# Autodesk Inventor assembly: Assembly1
(part 2 of 3)
- Mate:224: Plattform-Oberteil:1 ↔ DIN 125-1 B B 6,4:8
- Mate:225: Plattform-Oberteil:1 ↔ DIN 931-1 - replaced by DIN EN 24014 M6 x 30:4
- Mate:226: Plattform-Oberteil:1 ↔ DIN 931-1 - replaced by DIN EN 24014 M6 x 30:14
- Mate:227: Plattform-Oberteil:1 ↔ DIN 931-1 - replaced by DIN EN 24014 M6 x 30:5
- Mate:228: DIN 931-1 - replaced by DIN EN 24014 M8 x 45:1 ↔ DIN 125-1 B B 8,4:1
- Mate:229: DIN 931-1 - replaced by DIN EN 24014 M8 x 45:1 ↔ DIN 125-1 B B 8,4:1
- [Mate]: DIN 931-1 - replaced by DIN EN 24014 M8 x 45:2 ↔ DIN 125-1 B B 8,4:2
- [Mate]: DIN 931-1 - replaced by DIN EN 24014 M8 x 45:2 ↔ DIN 125-1 B B 8,4:2
- [Mate]: DIN 931-1 - replaced by DIN EN 24014 M8 x 45:3 ↔ DIN 125-1 B B 8,4:3
- [Mate]: DIN 931-1 - replaced by DIN EN 24014 M8 x 45:3 ↔ DIN 125-1 B B 8,4:3
- [Mate]: DIN 931-1 - replaced by DIN EN 24014 M8 x 45:4 ↔ DIN 125-1 B B 8,4:4
- [Mate]: DIN 931-1 - replaced by DIN EN 24014 M8 x 45:4 ↔ DIN 125-1 B B 8,4:4
- Mate:236: Plattform-Unterteil:1 ↔ DIN 125-1 B B 8,4:1
- Mate:237: Plattform-Unterteil:1 ↔ DIN 125-1 B B 8,4:4
- Mate:238: Plattform-Unterteil:1 ↔ DIN 125-1 B B 8,4:2
- Mate:239: Plattform-Unterteil:1 ↔ DIN 125-1 B B 8,4:3
- Mate:240: Verbindungsplatte:1 ↔ DIN 931-1 - replaced by DIN EN 24014 M8 x 45:3
- Mate:241: Verbindungsplatte:1 ↔ DIN 931-1 - replaced by DIN EN 24014 M8 x 45:4
- Mate:242: Plattform-Unterteil:1 ↔ DIN 931-1 - replaced by DIN EN 24014 M8 x 45:2
- Mate:243: Plattform-Unterteil:1 ↔ DIN 931-1 - replaced by DIN EN 24014 M8 x 45:1
- [Mate]: DIN 931-1 - replaced by DIN EN 24014 M8 x 50:5 ↔ DIN 125-1 B B 8,4:5
- [Mate]: DIN 931-1 - replaced by DIN EN 24014 M8 x 50:5 ↔ DIN 125-1 B B 8,4:5
- [Mate]: DIN 931-1 - replaced by DIN EN 24014 M8 x 50:6 ↔ DIN 125-1 B B 8,4:6
- [Mate]: DIN 931-1 - replaced by DIN EN 24014 M8 x 50:6 ↔ DIN 125-1 B B 8,4:6
- [Mate]: DIN 931-1 - replaced by DIN EN 24014 M8 x 50:7 ↔ DIN 125-1 B B 8,4:7
- [Mate]: DIN 931-1 - replaced by DIN EN 24014 M8 x 50:7 ↔ DIN 125-1 B B 8,4:7
- [Mate]: DIN 931-1 - replaced by DIN EN 24014 M8 x 50:8 ↔ DIN 125-1 B B 8,4:8
- [Mate]: DIN 931-1 - replaced by DIN EN 24014 M8 x 50:8 ↔ DIN 125-1 B B 8,4:8
- Mate:252: Verbindungsplatte:1 ↔ DIN 125-1 B B 8,4:8
- Mate:253: Verbindungsplatte:1 ↔ DIN 125-1 B B 8,4:7
- Mate:254: Verbindungsplatte:1 ↔ DIN 125-1 B B 8,4:6
- Mate:255: Verbindungsplatte:1 ↔ DIN 125-1 B B 8,4:5
- Mate:256: Verbindungsplatte:1 ↔ DIN 931-1 - replaced by DIN EN 24014 M8 x 50:8
- Mate:257: Verbindungsplatte:1 ↔ DIN 931-1 - replaced by DIN EN 24014 M8 x 50:7
- Mate:258: Verbindungsplatte:1 ↔ DIN 931-1 - replaced by DIN EN 24014 M8 x 50:6
- Mate:259: Verbindungsplatte:1 ↔ DIN 931-1 - replaced by DIN EN 24014 M8 x 50:5
- [Mate]: DIN 931-1 - replaced by DIN EN 24014 M6 x 50:3 ↔ DIN 125-1 B B 6,4:23
- [Mate]: DIN 931-1 - replaced by DIN EN 24014 M6 x 50:3 ↔ DIN 125-1 B B 6,4:23
- [Mate]: DIN 931-1 - replaced by DIN EN 24014 M6 x 50:2 ↔ DIN 125-1 B B 6,4:21
- [Mate]: DIN 931-1 - replaced by DIN EN 24014 M6 x 50:2 ↔ DIN 125-1 B B 6,4:21
- [Mate]: DIN 931-1 - replaced by DIN EN 24014 M6 x 50:1 ↔ DIN 125-1 B B 6,4:22
- [Mate]: DIN 931-1 - replaced by DIN EN 24014 M6 x 50:1 ↔ DIN 125-1 B B 6,4:22
- Mate:266: Deckel:1 ↔ DIN 125-1 B B 6,4:21
- Mate:267: Deckel:1 ↔ DIN 125-1 B B 6,4:22
- Mate:268: Deckel:1 ↔ DIN 125-1 B B 6,4:23
- Mate:269: Deckel:1 ↔ DIN 931-1 - replaced by DIN EN 24014 M6 x 50:2
- Mate:270: Deckel:1 ↔ DIN 931-1 - replaced by DIN EN 24014 M6 x 50:3
- Mate:271: Deckel:1 ↔ DIN 931-1 - replaced by DIN EN 24014 M6 x 50:1
- Mate:272: Festlagertopf:1 ↔ DIN 931-1 - replaced by DIN EN 24014 M6 x 50:2
- [Mate]: DIN 931-1 - replaced by DIN EN 24014 M5 x 25:1 ↔ DIN 125-1 B B 5,3:2
- [Mate]: DIN 931-1 - replaced by DIN EN 24014 M5 x 25:1 ↔ DIN 125-1 B B 5,3:2
- Mate:275: Verfahrschlitten:1 ↔ Gewindemutter:1
- Mate:276: Verfahrschlitten:1 ↔ Gewindemutter:1
- Mate:277: Verfahrschlitten:1 ↔ Gewindemutter:2
- Mate:278: Verfahrschlitten:1 ↔ Gewindemutter:2
- Mate:279: Verfahrschlitten:1 ↔ DIN 931-1 - replaced by DIN EN 24014 M5 x 25:1
- Mate:280: DIN 125-1 B B 5,3:2 ↔ Gewindemutter:1
- [Mate]: DIN 931-1 - replaced by DIN EN 24014 M5 x 25:2 ↔ DIN 125-1 B B 5,3:3
- [Mate]: DIN 931-1 - replaced by DIN EN 24014 M5 x 25:2 ↔ DIN 125-1 B B 5,3:3
- [Mate]: DIN 931-1 - replaced by DIN EN 24014 M5 x 25:3 ↔ DIN 125-1 B B 5,3:4
- [Mate]: DIN 931-1 - replaced by DIN EN 24014 M5 x 25:3 ↔ DIN 125-1 B B 5,3:4
- [Mate]: DIN 931-1 - replaced by DIN EN 24014 M5 x 25:4 ↔ DIN 125-1 B B 5,3:5
- [Mate]: DIN 931-1 - replaced by DIN EN 24014 M5 x 25:4 ↔ DIN 125-1 B B 5,3:5
- [Mate]: DIN 931-1 - replaced by DIN EN 24014 M5 x 25:5 ↔ DIN 125-1 B B 5,3:6
- [Mate]: DIN 931-1 - replaced by DIN EN 24014 M5 x 25:5 ↔ DIN 125-1 B B 5,3:6
- [Mate]: DIN 931-1 - replaced by DIN EN 24014 M5 x 25:6 ↔ DIN 125-1 B B 5,3:7
- [Mate]: DIN 931-1 - replaced by DIN EN 24014 M5 x 25:6 ↔ DIN 125-1 B B 5,3:7
- [Mate]: DIN 931-1 - replaced by DIN EN 24014 M5 x 25:7 ↔ DIN 125-1 B B 5,3:8
- [Mate]: DIN 931-1 - replaced by DIN EN 24014 M5 x 25:7 ↔ DIN 125-1 B B 5,3:8
- [Mate]: DIN 931-1 - replaced by DIN EN 24014 M5 x 25:8 ↔ DIN 125-1 B B 5,3:9
- [Mate]: DIN 931-1 - replaced by DIN EN 24014 M5 x 25:8 ↔ DIN 125-1 B B 5,3:9
- [Mate]: DIN 931-1 - replaced by DIN EN 24014 M5 x 25:9 ↔ DIN 125-1 B B 5,3:10
- [Mate]: DIN 931-1 - replaced by DIN EN 24014 M5 x 25:9 ↔ DIN 125-1 B B 5,3:10
- [Mate]: DIN 931-1 - replaced by DIN EN 24014 M5 x 25:11 ↔ DIN 125-1 B B 5,3:12
- [Mate]: DIN 931-1 - replaced by DIN EN 24014 M5 x 25:11 ↔ DIN 125-1 B B 5,3:12
- Mate:301: Verfahrschlitten:1 ↔ DIN 125-1 B B 5,3:9
- Mate:302: Verfahrschlitten:1 ↔ DIN 125-1 B B 5,3:10
- Mate:303: Verfahrschlitten:1 ↔ DIN 125-1 B B 5,3:12
- Mate:304: Verfahrschlitten:1 ↔ DIN 125-1 B B 5,3:7
- Mate:305: Verfahrschlitten:1 ↔ DIN 125-1 B B 5,3:5
- Mate:306: Gewindemutter:2 ↔ DIN 931-1 - replaced by DIN EN 24014 M5 x 25:11
- Mate:307: Gewindemutter:2 ↔ DIN 931-1 - replaced by DIN EN 24014 M5 x 25:6
- Mate:308: Gewindemutter:2 ↔ DIN 931-1 - replaced by DIN EN 24014 M5 x 25:4
- Mate:309: Gewindemutter:2 ↔ DIN 931-1 - replaced by DIN EN 24014 M5 x 25:8
- Mate:310: Gewindemutter:2 ↔ DIN 931-1 - replaced by DIN EN 24014 M5 x 25:9
- Mate:311: Verfahrschlitten:1 ↔ DIN 931-1 - replaced by DIN EN 24014 M5 x 25:8
- Mate:312: DIN 931-1 - replaced by DIN EN 24014 M5 x 25:1 ↔ Gewindemutter:1
- Mate:313: Verfahrschlitten:1 ↔ DIN 125-1 B B 5,3:6
- Mate:314: Verfahrschlitten:1 ↔ DIN 125-1 B B 5,3:8
- Mate:315: Verfahrschlitten:1 ↔ DIN 125-1 B B 5,3:4
- Mate:316: Verfahrschlitten:1 ↔ DIN 125-1 B B 5,3:3
- Mate:317: Gewindemutter:1 ↔ DIN 931-1 - replaced by DIN EN 24014 M5 x 25:7
- Mate:318: Gewindemutter:1 ↔ DIN 931-1 - replaced by DIN EN 24014 M5 x 25:3
- Mate:319: Gewindemutter:1 ↔ DIN 931-1 - replaced by DIN EN 24014 M5 x 25:5
- Mate:320: Gewindemutter:1 ↔ DIN 931-1 - replaced by DIN EN 24014 M5 x 25:2
- Mate:321: Festlagertopf:1 ↔ Führung:1
- Mate:322: Festlagertopf:1 ↔ Führung:2
- Mate:323: Festlagertopf:1 ↔ Führung:1
- Mate:324: Festlagertopf:1 ↔ Führung:2
- [Mate]: DIN 931-1 - replaced by DIN EN 24014 M5 x 50:4 ↔ DIN 125-1 B B 5,3:14
- [Mate]: DIN 931-1 - replaced by DIN EN 24014 M5 x 50:4 ↔ DIN 125-1 B B 5,3:14
- [Mate]: DIN 931-1 - replaced by DIN EN 24014 M5 x 50:1 ↔ DIN 125-1 B B 5,3:16
- [Mate]: DIN 931-1 - replaced by DIN EN 24014 M5 x 50:1 ↔ DIN 125-1 B B 5,3:16
- [Mate]: DIN 931-1 - replaced by DIN EN 24014 M5 x 50:2 ↔ DIN 125-1 B B 5,3:17
- [Mate]: DIN 931-1 - replaced by DIN EN 24014 M5 x 50:2 ↔ DIN 125-1 B B 5,3:17
- [Mate]: DIN 931-1 - replaced by DIN EN 24014 M5 x 50:5 ↔ DIN 125-1 B B 5,3:18
- [Mate]: DIN 931-1 - replaced by DIN EN 24014 M5 x 50:5 ↔ DIN 125-1 B B 5,3:18
- [Mate]: DIN 931-1 - replaced by DIN EN 24014 M5 x 50:6 ↔ DIN 125-1 B B 5,3:19
- [Mate]: DIN 931-1 - replaced by DIN EN 24014 M5 x 50:6 ↔ DIN 125-1 B B 5,3:19
- [Mate]: DIN 931-1 - replaced by DIN EN 24014 M5 x 50:3 ↔ DIN 125-1 B B 5,3:20
- [Mate]: DIN 931-1 - replaced by DIN EN 24014 M5 x 50:3 ↔ DIN 125-1 B B 5,3:20
- Mate:337: Festlagertopf:1 ↔ DIN 125-1 B B 5,3:14
- Mate:338: Festlagertopf:1 ↔ DIN 125-1 B B 5,3:16
- Mate:339: Festlagertopf:1 ↔ DIN 125-1 B B 5,3:19
- Mate:340: Festlagertopf:1 ↔ DIN 125-1 B B 5,3:17
- Mate:341: Festlagertopf:1 ↔ DIN 125-1 B B 5,3:20
- Mate:342: Festlagertopf:1 ↔ DIN 125-1 B B 5,3:18
- Mate:343: Festlagertopf:1 ↔ DIN 931-1 - replaced by DIN EN 24014 M5 x 50:5
- Mate:344: Festlagertopf:1 ↔ DIN 931-1 - replaced by DIN EN 24014 M5 x 50:6
- Mate:345: Festlagertopf:1 ↔ DIN 931-1 - replaced by DIN EN 24014 M5 x 50:4
- Mate:346: Festlagertopf:1 ↔ DIN 931-1 - replaced by DIN EN 24014 M5 x 50:3
- Mate:347: Festlagertopf:1 ↔ DIN 931-1 - replaced by DIN EN 24014 M5 x 50:1
- Mate:348: Festlagertopf:1 ↔ DIN 931-1 - replaced by DIN EN 24014 M5 x 50:2
- [Mate]: DIN 931-1 - replaced by DIN EN 24014 M5 x 25:12 ↔ DIN 125-1 B B 5,3:21
- [Mate]: DIN 931-1 - replaced by DIN EN 24014 M5 x 25:12 ↔ DIN 125-1 B B 5,3:21
- [Mate]: DIN 931-1 - replaced by DIN EN 24014 M5 x 25:13 ↔ DIN 125-1 B B 5,3:22
- [Mate]: DIN 931-1 - replaced by DIN EN 24014 M5 x 25:13 ↔ DIN 125-1 B B 5,3:22
- [Mate]: DIN 931-1 - replaced by DIN EN 24014 M5 x 25:14 ↔ DIN 125-1 B B 5,3:23
- [Mate]: DIN 931-1 - replaced by DIN EN 24014 M5 x 25:14 ↔ DIN 125-1 B B 5,3:23
- [Mate]: DIN 931-1 - replaced by DIN EN 24014 M5 x 25:15 ↔ DIN 125-1 B B 5,3:24
- [Mate]: DIN 931-1 - replaced by DIN EN 24014 M5 x 25:15 ↔ DIN 125-1 B B 5,3:24
- [Mate]: DIN 931-1 - replaced by DIN EN 24014 M5 x 25:16 ↔ DIN 125-1 B B 5,3:25
- [Mate]: DIN 931-1 - replaced by DIN EN 24014 M5 x 25:16 ↔ DIN 125-1 B B 5,3:25
- [Mate]: DIN 931-1 - replaced by DIN EN 24014 M5 x 25:17 ↔ DIN 125-1 B B 5,3:26
- [Mate]: DIN 931-1 - replaced by DIN EN 24014 M5 x 25:17 ↔ DIN 125-1 B B 5,3:26
- [Mate]: DIN 931-1 - replaced by DIN EN 24014 M5 x 25:18 ↔ DIN 125-1 B B 5,3:27
- [Mate]: DIN 931-1 - replaced by DIN EN 24014 M5 x 25:18 ↔ DIN 125-1 B B 5,3:27
- [Mate]: DIN 931-1 - replaced by DIN EN 24014 M5 x 25:19 ↔ DIN 125-1 B B 5,3:28
- [Mate]: DIN 931-1 - replaced by DIN EN 24014 M5 x 25:19 ↔ DIN 125-1 B B 5,3:28
- [Mate]: DIN 931-1 - replaced by DIN EN 24014 M5 x 25:20 ↔ DIN 125-1 B B 5,3:29
- [Mate]: DIN 931-1 - replaced by DIN EN 24014 M5 x 25:20 ↔ DIN 125-1 B B 5,3:29
- [Mate]: DIN 931-1 - replaced by DIN EN 24014 M5 x 25:21 ↔ DIN 125-1 B B 5,3:30
- [Mate]: DIN 931-1 - replaced by DIN EN 24014 M5 x 25:21 ↔ DIN 125-1 B B 5,3:30
- [Mate]: DIN 931-1 - replaced by DIN EN 24014 M5 x 25:22 ↔ DIN 125-1 B B 5,3:31
- [Mate]: DIN 931-1 - replaced by DIN EN 24014 M5 x 25:22 ↔ DIN 125-1 B B 5,3:31
- [Mate]: DIN 931-1 - replaced by DIN EN 24014 M5 x 25:23 ↔ DIN 125-1 B B 5,3:32
- [Mate]: DIN 931-1 - replaced by DIN EN 24014 M5 x 25:23 ↔ DIN 125-1 B B 5,3:32
- [Mate]: DIN 931-1 - replaced by DIN EN 24014 M5 x 25:24 ↔ DIN 125-1 B B 5,3:33
- [Mate]: DIN 931-1 - replaced by DIN EN 24014 M5 x 25:24 ↔ DIN 125-1 B B 5,3:33
- [Mate]: DIN 931-1 - replaced by DIN EN 24014 M5 x 25:25 ↔ DIN 125-1 B B 5,3:34
- [Mate]: DIN 931-1 - replaced by DIN EN 24014 M5 x 25:25 ↔ DIN 125-1 B B 5,3:34
- [Mate]: DIN 931-1 - replaced by DIN EN 24014 M5 x 25:26 ↔ DIN 125-1 B B 5,3:35
- [Mate]: DIN 931-1 - replaced by DIN EN 24014 M5 x 25:26 ↔ DIN 125-1 B B 5,3:35
- [Mate]: DIN 931-1 - replaced by DIN EN 24014 M5 x 25:27 ↔ DIN 125-1 B B 5,3:36
- [Mate]: DIN 931-1 - replaced by DIN EN 24014 M5 x 25:27 ↔ DIN 125-1 B B 5,3:36
- [Mate]: DIN 931-1 - replaced by DIN EN 24014 M5 x 25:28 ↔ DIN 125-1 B B 5,3:37
- [Mate]: DIN 931-1 - replaced by DIN EN 24014 M5 x 25:28 ↔ DIN 125-1 B B 5,3:37
- [Mate]: DIN 931-1 - replaced by DIN EN 24014 M5 x 25:29 ↔ DIN 125-1 B B 5,3:38
- [Mate]: DIN 931-1 - replaced by DIN EN 24014 M5 x 25:29 ↔ DIN 125-1 B B 5,3:38
- [Mate]: DIN 931-1 - replaced by DIN EN 24014 M5 x 25:30 ↔ DIN 125-1 B B 5,3:39
- [Mate]: DIN 931-1 - replaced by DIN EN 24014 M5 x 25:30 ↔ DIN 125-1 B B 5,3:39
- [Mate]: DIN 931-1 - replaced by DIN EN 24014 M5 x 25:31 ↔ DIN 125-1 B B 5,3:40
- [Mate]: DIN 931-1 - replaced by DIN EN 24014 M5 x 25:31 ↔ DIN 125-1 B B 5,3:40
- Mate:389: Verfahrschlitten:1 ↔ Führungsgleitlager:3
- Mate:390: Verfahrschlitten:1 ↔ Führungsgleitlager:4
- Mate:391: Führung:2 ↔ Führungsgleitlager:4
- Mate:393: Verfahrschlitten:1 ↔ Führungsgleitlager:3
- Mate:394: Verfahrschlitten:1 ↔ Führungsgleitlager:4
- Mate:395: Führungsgleitlager:3 ↔ DIN 125-1 B B 5,3:37
- Mate:396: Führungsgleitlager:3 ↔ DIN 125-1 B B 5,3:24
- Mate:397: Führungsgleitlager:3 ↔ DIN 125-1 B B 5,3:32
- Mate:398: Führungsgleitlager:3 ↔ DIN 125-1 B B 5,3:28
- Mate:399: Führungsgleitlager:3 ↔ DIN 125-1 B B 5,3:29
- Mate:400: Führungsgleitlager:3 ↔ DIN 125-1 B B 5,3:27
- Mate:401: Führungsgleitlager:3 ↔ DIN 125-1 B B 5,3:23
- Mate:402: Führungsgleitlager:3 ↔ DIN 125-1 B B 5,3:31
- Mate:403: Führungsgleitlager:3 ↔ DIN 125-1 B B 5,3:30
- Mate:404: Verfahrschlitten:1 ↔ DIN 125-1 B B 5,3:25
- Mate:405: Verfahrschlitten:1 ↔ DIN 931-1 - replaced by DIN EN 24014 M5 x 25:19
- Mate:406: Verfahrschlitten:1 ↔ DIN 931-1 - replaced by DIN EN 24014 M5 x 25:22
- Mate:407: Verfahrschlitten:1 ↔ DIN 931-1 - replaced by DIN EN 24014 M5 x 25:20
- Mate:408: Verfahrschlitten:1 ↔ DIN 931-1 - replaced by DIN EN 24014 M5 x 25:18
- Mate:409: Verfahrschlitten:1 ↔ DIN 931-1 - replaced by DIN EN 24014 M5 x 25:16
- Mate:410: Verfahrschlitten:1 ↔ DIN 931-1 - replaced by DIN EN 24014 M5 x 25:14
- Mate:411: Verfahrschlitten:1 ↔ DIN 931-1 - replaced by DIN EN 24014 M5 x 25:23
- Mate:412: Verfahrschlitten:1 ↔ DIN 931-1 - replaced by DIN EN 24014 M5 x 25:21
- Mate:413: Verfahrschlitten:1 ↔ DIN 931-1 - replaced by DIN EN 24014 M5 x 25:15
- Mate:414: Verfahrschlitten:1 ↔ DIN 931-1 - replaced by DIN EN 24014 M5 x 25:28
- Mate:415: Verfahrschlitten:1 ↔ Führungsgleitlager:2
- Mate:416: Führung:2 ↔ Führungsgleitlager:2
- Mate:417: Führung:1 ↔ Führungsgleitlager:1
- Mate:418: Verfahrschlitten:1 ↔ Führungsgleitlager:1
- Mate:420: Verfahrschlitten:1 ↔ Führungsgleitlager:2
- Mate:421: Verfahrschlitten:1 ↔ DIN 125-1 B B 5,3:21
- Mate:422: Verfahrschlitten:1 ↔ DIN 125-1 B B 5,3:34
- Mate:423: Verfahrschlitten:1 ↔ DIN 125-1 B B 5,3:36
- Mate:424: Verfahrschlitten:1 ↔ DIN 125-1 B B 5,3:26
- Mate:425: Verfahrschlitten:1 ↔ DIN 125-1 B B 5,3:38
- Mate:426: Verfahrschlitten:1 ↔ DIN 125-1 B B 5,3:40
- Mate:427: Verfahrschlitten:1 ↔ DIN 125-1 B B 5,3:33
- Mate:428: Verfahrschlitten:1 ↔ DIN 125-1 B B 5,3:22
- Mate:429: Verfahrschlitten:1 ↔ DIN 125-1 B B 5,3:39
- Mate:430: Verfahrschlitten:1 ↔ DIN 125-1 B B 5,3:35
- Mate:431: Führungsgleitlager:1 ↔ DIN 931-1 - replaced by DIN EN 24014 M5 x 25:31
- Mate:432: Führungsgleitlager:1 ↔ DIN 931-1 - replaced by DIN EN 24014 M5 x 25:26
- Mate:433: Führungsgleitlager:1 ↔ DIN 931-1 - replaced by DIN EN 24014 M5 x 25:27
- Mate:434: Führungsgleitlager:1 ↔ DIN 931-1 - replaced by DIN EN 24014 M5 x 25:29
- Mate:435: Führungsgleitlager:2 ↔ DIN 931-1 - replaced by DIN EN 24014 M5 x 25:17
- Mate:436: Führungsgleitlager:2 ↔ DIN 931-1 - replaced by DIN EN 24014 M5 x 25:25
- Mate:437: Führungsgleitlager:2 ↔ DIN 931-1 - replaced by DIN EN 24014 M5 x 25:13
- Mate:438: DIN 931-1 - replaced by DIN EN 24014 M5 x 25:12 ↔ Führungsgleitlager:2
- Mate:439: Führungsgleitlager:2 ↔ DIN 931-1 - replaced by DIN EN 24014 M5 x 25:24
- Mate:440: Führungsgleitlager:1 ↔ DIN 931-1 - replaced by DIN EN 24014 M5 x 25:30
- Flush:4: Festlagertopf:1 ↔ Grundplatte:1
- Mate:447: Festlagertopf:1 ↔ Grundplatte:1
- [Mate]: DIN 931-1 - replaced by DIN EN 24014 M12 x 70:1 ↔ DIN 125-1 B B 13:1
- [Mate]: DIN 931-1 - replaced by DIN EN 24014 M12 x 70:1 ↔ DIN 125-1 B B 13:1
- [Mate]: DIN 931-1 - replaced by DIN EN 24014 M12 x 70:2 ↔ DIN 125-1 B B 13:2
- [Mate]: DIN 931-1 - replaced by DIN EN 24014 M12 x 70:2 ↔ DIN 125-1 B B 13:2
- [Mate]: DIN 931-1 - replaced by DIN EN 24014 M12 x 70:3 ↔ DIN 125-1 B B 13:3
- [Mate]: DIN 931-1 - replaced by DIN EN 24014 M12 x 70:3 ↔ DIN 125-1 B B 13:3
- [Mate]: DIN 931-1 - replaced by DIN EN 24014 M12 x 70:4 ↔ DIN 125-1 B B 13:4
- [Mate]: DIN 931-1 - replaced by DIN EN 24014 M12 x 70:4 ↔ DIN 125-1 B B 13:4
- [Mate]: DIN 931-1 - replaced by DIN EN 24014 M12 x 70:5 ↔ DIN 125-1 B B 13:5
- [Mate]: DIN 931-1 - replaced by DIN EN 24014 M12 x 70:5 ↔ DIN 125-1 B B 13:5
- [Mate]: DIN 931-1 - replaced by DIN EN 24014 M12 x 70:6 ↔ DIN 125-1 B B 13:6
- [Mate]: DIN 931-1 - replaced by DIN EN 24014 M12 x 70:6 ↔ DIN 125-1 B B 13:6
- [Mate]: DIN 931-1 - replaced by DIN EN 24014 M12 x 70:7 ↔ DIN 125-1 B B 13:7
- [Mate]: DIN 931-1 - replaced by DIN EN 24014 M12 x 70:7 ↔ DIN 125-1 B B 13:7
- [Mate]: DIN 931-1 - replaced by DIN EN 24014 M12 x 70:8 ↔ DIN 125-1 B B 13:8
- [Mate]: DIN 931-1 - replaced by DIN EN 24014 M12 x 70:8 ↔ DIN 125-1 B B 13:8
- Mate:465: Grundplatte:1 ↔ DIN 125-1 B B 13:1
- Mate:466: Grundplatte:1 ↔ DIN 125-1 B B 13:2
- Mate:467: Grundplatte:1 ↔ DIN 125-1 B B 13:3
- Mate:468: Grundplatte:1 ↔ DIN 125-1 B B 13:4
- Mate:469: Grundplatte:1 ↔ DIN 125-1 B B 13:5
- Mate:470: Grundplatte:1 ↔ DIN 125-1 B B 13:6
- Mate:471: Grundplatte:1 ↔ DIN 125-1 B B 13:7
- Mate:472: Grundplatte:1 ↔ DIN 125-1 B B 13:8
- Mate:473: Festlagertopf:1 ↔ DIN 931-1 - replaced by DIN EN 24014 M12 x 70:3
- Mate:474: Festlagertopf:1 ↔ DIN 931-1 - replaced by DIN EN 24014 M12 x 70:4
- Mate:475: Festlagertopf:1 ↔ DIN 931-1 - replaced by DIN EN 24014 M12 x 70:5
- Mate:476: Festlagertopf:1 ↔ DIN 931-1 - replaced by DIN EN 24014 M12 x 70:6
- Mate:477: Festlagertopf:1 ↔ DIN 931-1 - replaced by DIN EN 24014 M12 x 70:7
- Mate:478: Festlagertopf:1 ↔ DIN 931-1 - replaced by DIN EN 24014 M12 x 70:1
- Mate:479: Festlagertopf:1 ↔ DIN 931-1 - replaced by DIN EN 24014 M12 x 70:8
- [Mate]: DIN 931-1 - replaced by DIN EN 24014 M12 x 70:9 ↔ DIN 125-1 B B 13:9
- [Mate]: DIN 931-1 - replaced by DIN EN 24014 M12 x 70:9 ↔ DIN 125-1 B B 13:9
- [Mate]: DIN 931-1 - replaced by DIN EN 24014 M12 x 70:10 ↔ DIN 125-1 B B 13:10
- [Mate]: DIN 931-1 - replaced by DIN EN 24014 M12 x 70:10 ↔ DIN 125-1 B B 13:10
- [Mate]: DIN 931-1 - replaced by DIN EN 24014 M12 x 70:11 ↔ DIN 125-1 B B 13:11
- [Mate]: DIN 931-1 - replaced by DIN EN 24014 M12 x 70:11 ↔ DIN 125-1 B B 13:11
- [Mate]: DIN 931-1 - replaced by DIN EN 24014 M12 x 70:12 ↔ DIN 125-1 B B 13:12
- [Mate]: DIN 931-1 - replaced by DIN EN 24014 M12 x 70:12 ↔ DIN 125-1 B B 13:12
- Mate:488: Grundplatte:1 ↔ DIN 125-1 B B 13:10
- Mate:489: Grundplatte:1 ↔ DIN 125-1 B B 13:9
- Mate:490: Grundplatte:1 ↔ DIN 125-1 B B 13:11
- Mate:491: Grundplatte:1 ↔ DIN 125-1 B B 13:12
- Mate:492: Loslagertopf:1 ↔ DIN 931-1 - replaced by DIN EN 24014 M12 x 70:10
- Mate:493: Loslagertopf:1 ↔ DIN 931-1 - replaced by DIN EN 24014 M12 x 70:11
- Mate:494: Loslagertopf:1 ↔ DIN 931-1 - replaced by DIN EN 24014 M12 x 70:9
- Mate:495: Loslagertopf:1 ↔ DIN 931-1 - replaced by DIN EN 24014 M12 x 70:12
- Mate:496: Federwellen-Gleitlager:10 ↔ Federführungswellen:5
- Mate:497 (30 mm): Plattform-Oberteil:1 ↔ Plattform-Unterteil:1
- Mate:499: Grundplatte:1 ↔ DIN 931-1 - replaced by DIN EN 24014 M12 x 70:11
- Mate:500: Grundplatte:1 ↔ DIN 931-1 - replaced by DIN EN 24014 M12 x 70:2
- Mate:501: Verfahrschlitten:1 ↔ Schutzpuffer:2
- Mate:502: Verfahrschlitten:1 ↔ Schutzpuffer:1
- Angle:18 (0 deg): Verfahrschlitten:1 ↔ Schutzpuffer:1
- Angle:19 (0 deg): Verfahrschlitten:1 ↔ Schutzpuffer:2
- Flush:5 (-5 mm): Verfahrschlitten:1 ↔ Schutzpuffer:1
- Flush:6 (-5 mm): Verfahrschlitten:1 ↔ Schutzpuffer:1
- Flush:7 (-5 mm): Verfahrschlitten:1 ↔ Schutzpuffer:2
- Flush:8 (-5 mm): Verfahrschlitten:1 ↔ Schutzpuffer:2
- Mate:504: Verfahrschlitten:1 ↔ DIN 931-1 - replaced by DIN EN 24014 M5 x 25:26
- Mate:505: Führung:1 ↔ Führungsgleitlager:3
- Angle:20 (0 deg): Grundplatte:1 ↔ Elektromotor:1
- Flush:9 (15 mm): Grundplatte:1 ↔ Elektromotor:1
- Mate:508: DIN 912 - replaced by DIN EN ISO 4762 M12 x 50:1 ↔ DIN 125-1 B B 13:13
- Mate:509: DIN 912 - replaced by DIN EN ISO 4762 M12 x 50:1 ↔ DIN 125-1 B B 13:13
- [Mate]: DIN 912 - replaced by DIN EN ISO 4762 M12 x 50:2 ↔ DIN 125-1 B B 13:14
- [Mate]: DIN 912 - replaced by DIN EN ISO 4762 M12 x 50:2 ↔ DIN 125-1 B B 13:14
- [Mate]: DIN 912 - replaced by DIN EN ISO 4762 M12 x 50:3 ↔ DIN 125-1 B B 13:15
- [Mate]: DIN 912 - replaced by DIN EN ISO 4762 M12 x 50:3 ↔ DIN 125-1 B B 13:15
- [Mate]: DIN 912 - replaced by DIN EN ISO 4762 M12 x 50:4 ↔ DIN 125-1 B B 13:16
- [Mate]: DIN 912 - replaced by DIN EN ISO 4762 M12 x 50:4 ↔ DIN 125-1 B B 13:16
- [Mate]: DIN 912 - replaced by DIN EN ISO 4762 M12 x 50:5 ↔ DIN 125-1 B B 13:17
- [Mate]: DIN 912 - replaced by DIN EN ISO 4762 M12 x 50:5 ↔ DIN 125-1 B B 13:17
- [Mate]: DIN 912 - replaced by DIN EN ISO 4762 M12 x 50:6 ↔ DIN 125-1 B B 13:18
- [Mate]: DIN 912 - replaced by DIN EN ISO 4762 M12 x 50:6 ↔ DIN 125-1 B B 13:18
- Mate:520: Grundplatte:1 ↔ DIN 125-1 B B 13:15
- Mate:521: Grundplatte:1 ↔ DIN 125-1 B B 13:17
- Mate:522: Grundplatte:1 ↔ DIN 125-1 B B 13:15
- Mate:523: Grundplatte:1 ↔ DIN 125-1 B B 13:17
- Mate:524: Grundplatte:1 ↔ DIN 125-1 B B 13:14
- Mate:525: Grundplatte:1 ↔ DIN 125-1 B B 13:13
- Mate:526: Elektromotor:1 ↔ DIN 912 - replaced by DIN EN ISO 4762 M12 x 50:6
- Mate:527: Elektromotor:1 ↔ DIN 912 - replaced by DIN EN ISO 4762 M12 x 50:3
- Mate:528: Elektromotor:1 ↔ DIN 912 - replaced by DIN EN ISO 4762 M12 x 50:5
- Mate:529: Elektromotor:1 ↔ DIN 912 - replaced by DIN EN ISO 4762 M12 x 50:2
- Mate:530: Elektromotor:1 ↔ DIN 912 - replaced by DIN EN ISO 4762 M12 x 50:1
- Mate:531: Grundplatte:1 ↔ DIN 125-1 B B 13:18
- Mate:532: Grundplatte:1 ↔ DIN 125-1 B B 13:16
- Mate:533: Elektromotor:1 ↔ DIN 912 - replaced by DIN EN ISO 4762 M12 x 50:4
- Mate:534: Elektromotor:1 ↔ DIN 125-1 B B 13:24
- Mate:535: Elektromotor:1 ↔ DIN 125-1 B B 13:23
- Mate:536: Elektromotor:1 ↔ DIN 125-1 B B 13:22
- Mate:537: Elektromotor:1 ↔ DIN 125-1 B B 13:21
- Mate:538: Elektromotor:1 ↔ DIN 125-1 B B 13:20
- Mate:539: Elektromotor:1 ↔ DIN 125-1 B B 13:19
- Mate:540: DIN 912 - replaced by DIN EN ISO 4762 M12 x 50:3 ↔ DIN 125-1 B B 13:22
- Mate:541: DIN 912 - replaced by DIN EN ISO 4762 M12 x 50:5 ↔ DIN 125-1 B B 13:19
- Mate:542: DIN 912 - replaced by DIN EN ISO 4762 M12 x 50:6 ↔ DIN 125-1 B B 13:20
- Mate:543: DIN 912 - replaced by DIN EN ISO 4762 M12 x 50:2 ↔ DIN 125-1 B B 13:21
- Mate:544: DIN 912 - replaced by DIN EN ISO 4762 M12 x 50:1 ↔ DIN 125-1 B B 13:24
- Mate:545: DIN 912 - replaced by DIN EN ISO 4762 M12 x 50:4 ↔ DIN 125-1 B B 13:23
- Insert:1: DIN 125-1 B B 13:21 ↔ DIN 6915 M12:1
- Insert:2: DIN 125-1 B B 13:24 ↔ DIN 6915 M12:2
- Insert:3: DIN 125-1 B B 13:23 ↔ DIN 6915 M12:3
- Insert:4: DIN 125-1 B B 13:20 ↔ DIN 6915 M12:4
- Insert:5: DIN 125-1 B B 13:19 ↔ DIN 6915 M12:5
- Insert:6: DIN 125-1 B B 13:22 ↔ DIN 6915 M12:6
- Mate:546: Grundplatte:1 ↔ DIN 912 - replaced by DIN EN ISO 4762 M12 x 50:6
- Mate:547: Grundplatte:1 ↔ Elektromotor:1
- Mate:548: Spindel:1 ↔ Elektromotor:1
- Mate:549: Elektromotor:1 ↔ Ausgleichskupplung:1
- Mate:550: Elektromotor:1 ↔ Ausgleichskupplung:1
- Mate:551: Spindel:1 ↔ DIN 6885-1 A A 4 x 4 x 12:1
- Mate:552: Spindel:1 ↔ DIN 6885-1 A A 4 x 4 x 12:1
- Mate:553: Spindel:1 ↔ DIN 6885-1 A A 4 x 4 x 12:1
- Angle:21 (0 deg): Spindel:1 ↔ Festlagertopf:1
- Angle:22 (0 deg): Ausgleichskupplung:1 ↔ DIN 6885-1 A A 4 x 4 x 12:1
- Mate:557: DIN EN ISO 4026 M8 x 10:1 ↔ Rubber Kupplung:1
- Mate:558: DIN EN ISO 4026 M8 x 10:2 ↔ Rubber Kupplung:2
- Mate:559: DIN EN ISO 4026 M8 x 10:1 ↔ Rubber Kupplung:1
- Mate:560: DIN EN ISO 4026 M8 x 10:2 ↔ Rubber Kupplung:2
- Mate:561: Ausgleichskupplung:1 ↔ DIN EN ISO 4026 M8 x 10:2
- Mate:562: Ausgleichskupplung:1 ↔ DIN EN ISO 4026 M8 x 10:1
- Mate:563: DIN 6885-1 A A 4 x 4 x 12:2 ↔ Rubber Kupplung:1
- Mate:564: DIN 6885-1 A A 4 x 4 x 12:1 ↔ Rubber Kupplung:2
- Mate:617: Plattform-Unterteil:1 ↔ Elektrischer Schalter:1
- Mate:618: Plattform-Unterteil:1 ↔ Elektrischer Schalter:2
- Flush:10 (175 mm): Plattform-Unterteil:1 ↔ Elektrischer Schalter:2
- Flush:11 (-475 mm): Plattform-Unterteil:1 ↔ Elektrischer Schalter:1
- Flush:12 (-25 mm): Plattform-Unterteil:1 ↔ Elektrischer Schalter:2
- Flush:13 (25 mm): Plattform-Unterteil:1 ↔ Elektrischer Schalter:1
- Mate:619: Grundplatte:1 ↔ Wand:1
- [Mate]: DIN 931-1 - replaced by DIN EN 24014 M12 x 55:4 ↔ DIN 125-1 B B 13:26
- [Mate]: DIN 931-1 - replaced by DIN EN 24014 M12 x 55:4 ↔ DIN 125-1 B B 13:26
- [Mate]: DIN 931-1 - replaced by DIN EN 24014 M12 x 55:3 ↔ DIN 125-1 B B 13:25
- [Mate]: DIN 931-1 - replaced by DIN EN 24014 M12 x 55:3 ↔ DIN 125-1 B B 13:25
- [Mate]: DIN 931-1 - replaced by DIN EN 24014 M12 x 55:1 ↔ DIN 125-1 B B 13:28
- [Mate]: DIN 931-1 - replaced by DIN EN 24014 M12 x 55:1 ↔ DIN 125-1 B B 13:28
- [Mate]: DIN 931-1 - replaced by DIN EN 24014 M12 x 55:2 ↔ DIN 125-1 B B 13:27
- [Mate]: DIN 931-1 - replaced by DIN EN 24014 M12 x 55:2 ↔ DIN 125-1 B B 13:27
- Mate:628: Grundplatte:1 ↔ DIN 125-1 B B 13:28
- Mate:629: Grundplatte:1 ↔ DIN 125-1 B B 13:27
- Mate:630: Grundplatte:1 ↔ DIN 125-1 B B 13:25
- Mate:631: Grundplatte:1 ↔ DIN 125-1 B B 13:26
- Mate:632: Grundplatte:1 ↔ DIN 931-1 - replaced by DIN EN 24014 M12 x 55:4
- Mate:633: Grundplatte:1 ↔ DIN 931-1 - replaced by DIN EN 24014 M12 x 55:3
- Mate:634: Grundplatte:1 ↔ DIN 931-1 - replaced by DIN EN 24014 M12 x 55:2
- Mate:635: Grundplatte:1 ↔ DIN 931-1 - replaced by DIN EN 24014 M12 x 55:1
- Mate:636: Elektromotor:1 ↔ DIN 6885-1 A A 4 x 4 x 12:2
- Mate:637: Elektromotor:1 ↔ DIN 6885-1 A A 4 x 4 x 12:2
- Mate:638: Elektromotor:1 ↔ DIN 6885-1 A A 4 x 4 x 12:2
- Angle:23 (0 deg): DIN 6885-1 A A 4 x 4 x 12:2 ↔ Rubber Kupplung:1
- Angle:24 (0 deg): DIN 6885-1 A A 4 x 4 x 12:1 ↔ Rubber Kupplung:2
- Mate:639: Federführungswellen:2 ↔ Compress Spring1:1
- Mate:640: Federführungswellen:4 ↔ Compress Spring1:2
- Mate:641: Federführungswellen:5 ↔ Compress Spring1:3
- Mate:642: Federführungswellen:6 ↔ Compress Spring1:4
- Mate:643: Federführungswellen:3 ↔ Compress Spring1:5
- Mate:644: Federführungswellen:1 ↔ Compress Spring1:6
- Mate:645: Plattform-Oberteil:1 ↔ Compress Spring1:1
- Mate:646: Plattform-Oberteil:1 ↔ Compress Spring1:6
- Mate:647: Plattform-Oberteil:1 ↔ Compress Spring1:2
- Mate:648: Plattform-Oberteil:1 ↔ Compress Spring1:3
- Mate:649: Plattform-Oberteil:1 ↔ Compress Spring1:4
- Mate:650: Plattform-Oberteil:1 ↔ Compress Spring1:5
- Mate:651: DIN 625 SKF- with two RS1 seals SKF 6206-2RS1:1 ↔ DIN 5406 Type MB/MBL (->DIN 981) MB6:1
- Mate:652: DIN 625 SKF- with two RS1 seals SKF 6005-2RSH:1 ↔ DIN 5406 Type MB/MBL (->DIN 981) MB5:1
- Angle:25 (0 deg): DIN 931-1 - replaced by DIN EN 24014 M5 x 50:4 ↔ Grundplatte:1
- Angle:26 (0 deg): DIN 931-1 - replaced by DIN EN 24014 M5 x 50:5 ↔ Grundplatte:1
- Angle:27 (0 deg): DIN 931-1 - replaced by DIN EN 24014 M5 x 50:6 ↔ Grundplatte:1
- Angle:28 (0 deg): DIN 931-1 - replaced by DIN EN 24014 M6 x 50:1 ↔ Grundplatte:1
- Angle:29 (0 deg): DIN 931-1 - replaced by DIN EN 24014 M5 x 50:2 ↔ Grundplatte:1
- Angle:30 (0 deg): DIN 931-1 - replaced by DIN EN 24014 M5 x 50:1 ↔ Grundplatte:1
- Mate:653: Führung:1 ↔ DIN 931-1 - replaced by DIN EN 24014 M5 x 50:1
- Angle:31 (0 deg): DIN 931-1 - replaced by DIN EN 24014 M6 x 50:1 ↔ Grundplatte:1
- Angle:32 (0 deg): DIN 931-1 - replaced by DIN EN 24014 M6 x 50:3 ↔ Grundplatte:1
- Angle:33 (0 deg): DIN 931-1 - replaced by DIN EN 24014 M6 x 50:2 ↔ Grundplatte:1
- Angle:34 (0 deg): Grundplatte:1 ↔ DIN 6915 M12:3
- Angle:35 (0 deg): Grundplatte:1 ↔ DIN 6915 M12:2
- Angle:36 (0 deg): Grundplatte:1 ↔ DIN 6915 M12:1
- Angle:37 (0 deg): Grundplatte:1 ↔ DIN 912 - replaced by DIN EN ISO 4762 M12 x 50:1
- Angle:38 (0 deg): Grundplatte:1 ↔ DIN 912 - replaced by DIN EN ISO 4762 M12 x 50:4
- Angle:39 (0 deg): Grundplatte:1 ↔ DIN 912 - replaced by DIN EN ISO 4762 M12 x 50:2
- Angle:40 (0 deg): Grundplatte:1 ↔ DIN 6915 M12:6
- Angle:41 (0 deg): Grundplatte:1 ↔ DIN 6915 M12:5
- Angle:42 (0 deg): Grundplatte:1 ↔ DIN 6915 M12:4
- Angle:43 (0 deg): Grundplatte:1 ↔ DIN 912 - replaced by DIN EN ISO 4762 M12 x 50:6
- Angle:44 (0 deg): Grundplatte:1 ↔ DIN 912 - replaced by DIN EN ISO 4762 M12 x 50:5
- Angle:45 (0 deg): Grundplatte:1 ↔ DIN 912 - replaced by DIN EN ISO 4762 M12 x 50:3
- Angle:82 (0 deg): DIN 931-1 - replaced by DIN EN 24014 M12 x 70:11 ↔ DIN EN ISO 4026 M8 x 10:2
- Angle:83 (0 deg): DIN 931-1 - replaced by DIN EN 24014 M12 x 70:11 ↔ DIN EN ISO 4026 M8 x 10:1
- Angle:84 (0 deg): Verfahrschlitten:1 ↔ DIN 931-1 - replaced by DIN EN 24014 M12 x 55:2
- Angle:85 (0 deg): Verfahrschlitten:1 ↔ DIN 931-1 - replaced by DIN EN 24014 M12 x 55:1
- Angle:86 (0 deg): Grundplatte:1 ↔ DIN 931-1 - replaced by DIN EN 24014 M12 x 70:10
- Angle:87 (0 deg): Grundplatte:1 ↔ DIN 931-1 - replaced by DIN EN 24014 M12 x 70:11
- Angle:88 (0 deg): Grundplatte:1 ↔ DIN 931-1 - replaced by DIN EN 24014 M12 x 70:9
- Angle:89 (0 deg): Grundplatte:1 ↔ DIN 931-1 - replaced by DIN EN 24014 M12 x 70:12
- Angle:90 (0 deg): Grundplatte:1 ↔ DIN 931-1 - replaced by DIN EN 24014 M12 x 70:8
- Angle:91 (0 deg): Grundplatte:1 ↔ DIN 931-1 - replaced by DIN EN 24014 M12 x 70:2
- Angle:92 (0 deg): Grundplatte:1 ↔ DIN 931-1 - replaced by DIN EN 24014 M12 x 70:1
- Angle:93 (0 deg): Grundplatte:1 ↔ DIN 931-1 - replaced by DIN EN 24014 M12 x 70:7
- Angle:94 (0 deg): Grundplatte:1 ↔ DIN 931-1 - replaced by DIN EN 24014 M12 x 70:6
- Angle:95 (0 deg): Grundplatte:1 ↔ DIN 931-1 - replaced by DIN EN 24014 M12 x 70:5
- Angle:96 (0 deg): Grundplatte:1 ↔ DIN 931-1 - replaced by DIN EN 24014 M12 x 70:4
- Angle:97 (0 deg): Grundplatte:1 ↔ DIN 931-1 - replaced by DIN EN 24014 M12 x 70:3
- Angle:102 (0 deg): Verfahrschlitten:1 ↔ DIN 931-1 - replaced by DIN EN 24014 M5 x 25:24
- Angle:103 (0 deg): Verfahrschlitten:1 ↔ DIN 931-1 - replaced by DIN EN 24014 M5 x 25:13
- Angle:104 (0 deg): DIN 931-1 - replaced by DIN EN 24014 M5 x 25:12 ↔ DIN 931-1 - replaced by DIN EN 24014 M5 x 25:24
- Angle:105 (0 deg): DIN 931-1 - replaced by DIN EN 24014 M5 x 25:12 ↔ DIN 931-1 - replaced by DIN EN 24014 M5 x 25:17
- Angle:106 (0 deg): DIN 931-1 - replaced by DIN EN 24014 M5 x 25:13 ↔ DIN 931-1 - replaced by DIN EN 24014 M5 x 25:25
- Angle:107 (0 deg): Verfahrschlitten:1 ↔ DIN 931-1 - replaced by DIN EN 24014 M5 x 25:5
- Angle:108 (0 deg): DIN 931-1 - replaced by DIN EN 24014 M5 x 25:3 ↔ DIN 931-1 - replaced by DIN EN 24014 M5 x 25:5
- Angle:109 (0 deg): DIN 931-1 - replaced by DIN EN 24014 M5 x 25:2 ↔ DIN 931-1 - replaced by DIN EN 24014 M5 x 25:5
- Angle:110 (0 deg): DIN 931-1 - replaced by DIN EN 24014 M5 x 25:5 ↔ DIN 931-1 - replaced by DIN EN 24014 M5 x 25:7
- Angle:111 (0 deg): DIN 931-1 - replaced by DIN EN 24014 M5 x 25:1 ↔ DIN 931-1 - replaced by DIN EN 24014 M5 x 25:2
- Angle:112 (0 deg): Verfahrschlitten:1 ↔ DIN 931-1 - replaced by DIN EN 24014 M5 x 25:30
- Angle:113 (0 deg): DIN 931-1 - replaced by DIN EN 24014 M5 x 25:29 ↔ DIN 931-1 - replaced by DIN EN 24014 M5 x 25:30
- Angle:114 (0 deg): DIN 931-1 - replaced by DIN EN 24014 M5 x 25:30 ↔ DIN 931-1 - replaced by DIN EN 24014 M5 x 25:31
- Angle:115 (0 deg): DIN 931-1 - replaced by DIN EN 24014 M5 x 25:26 ↔ DIN 931-1 - replaced by DIN EN 24014 M5 x 25:30
- Angle:116 (0 deg): DIN 931-1 - replaced by DIN EN 24014 M5 x 25:27 ↔ DIN 931-1 - replaced by DIN EN 24014 M5 x 25:30
- Angle:117 (0 deg): Verfahrschlitten:1 ↔ DIN 931-1 - replaced by DIN EN 24014 M5 x 25:20
- Angle:118 (0 deg): DIN 931-1 - replaced by DIN EN 24014 M5 x 25:15 ↔ DIN 931-1 - replaced by DIN EN 24014 M5 x 25:20
- Angle:119 (0 deg): DIN 931-1 - replaced by DIN EN 24014 M5 x 25:19 ↔ DIN 931-1 - replaced by DIN EN 24014 M5 x 25:20
- Angle:120 (0 deg): DIN 931-1 - replaced by DIN EN 24014 M5 x 25:20 ↔ DIN 931-1 - replaced by DIN EN 24014 M5 x 25:22
- Angle:121 (0 deg): DIN 931-1 - replaced by DIN EN 24014 M5 x 25:18 ↔ DIN 931-1 - replaced by DIN EN 24014 M5 x 25:20
- Angle:122 (0 deg): Verfahrschlitten:1 ↔ DIN 931-1 - replaced by DIN EN 24014 M5 x 25:11
- Angle:123 (0 deg): DIN 931-1 - replaced by DIN EN 24014 M5 x 25:9 ↔ DIN 931-1 - replaced by DIN EN 24014 M5 x 25:11
- Angle:124 (0 deg): DIN 931-1 - replaced by DIN EN 24014 M5 x 25:8 ↔ DIN 931-1 - replaced by DIN EN 24014 M5 x 25:11
- Angle:125 (0 deg): DIN 931-1 - replaced by DIN EN 24014 M5 x 25:6 ↔ DIN 931-1 - replaced by DIN EN 24014 M5 x 25:11
- Angle:126 (0 deg): Verfahrschlitten:1 ↔ DIN 931-1 - replaced by DIN EN 24014 M5 x 25:4
- Angle:127 (0 deg): Verfahrschlitten:1 ↔ DIN 931-1 - replaced by DIN EN 24014 M5 x 25:28
- Angle:128 (0 deg): DIN 931-1 - replaced by DIN EN 24014 M5 x 25:14 ↔ DIN 931-1 - replaced by DIN EN 24014 M5 x 25:28
- Angle:129 (0 deg): DIN 931-1 - replaced by DIN EN 24014 M5 x 25:21 ↔ DIN 931-1 - replaced by DIN EN 24014 M5 x 25:28
- Angle:130 (0 deg): DIN 931-1 - replaced by DIN EN 24014 M5 x 25:16 ↔ DIN 931-1 - replaced by DIN EN 24014 M5 x 25:28
- Angle:131 (0 deg): DIN 931-1 - replaced by DIN EN 24014 M5 x 25:23 ↔ DIN 931-1 - replaced by DIN EN 24014 M5 x 25:28
- Angle:136 (0 deg): Plattform-Unterteil:1 ↔ DIN 931-1 - replaced by DIN EN 24014 M6 x 30:19
- Angle:137 (0 deg): DIN 931-1 - replaced by DIN EN 24014 M6 x 30:19 ↔ DIN 931-1 - replaced by DIN EN 24014 M6 x 30:20
- Angle:138 (0 deg): DIN 931-1 - replaced by DIN EN 24014 M6 x 30:16 ↔ DIN 931-1 - replaced by DIN EN 24014 M6 x 30:20
- Angle:139 (0 deg): DIN 931-1 - replaced by DIN EN 24014 M6 x 30:2 ↔ DIN 931-1 - replaced by DIN EN 24014 M6 x 30:16
- Angle:140 (0 deg): DIN 931-1 - replaced by DIN EN 24014 M6 x 30:2 ↔ DIN 931-1 - replaced by DIN EN 24014 M6 x 30:17
- Angle:141 (0 deg): DIN 931-1 - replaced by DIN EN 24014 M6 x 30:1 ↔ DIN 931-1 - replaced by DIN EN 24014 M6 x 30:2
- Angle:142 (0 deg): DIN 931-1 - replaced by DIN EN 24014 M6 x 30:2 ↔ DIN 931-1 - replaced by DIN EN 24014 M6 x 30:7
- Angle:143 (0 deg): DIN 931-1 - replaced by DIN EN 24014 M6 x 30:7 ↔ DIN 931-1 - replaced by DIN EN 24014 M6 x 30:8
- Angle:144 (0 deg): DIN 931-1 - replaced by DIN EN 24014 M6 x 30:8 ↔ DIN 931-1 - replaced by DIN EN 24014 M6 x 30:18
- Angle:145 (0 deg): DIN 931-1 - replaced by DIN EN 24014 M6 x 30:10 ↔ DIN 931-1 - replaced by DIN EN 24014 M6 x 30:18
- Angle:146 (0 deg): DIN 931-1 - replaced by DIN EN 24014 M6 x 30:10 ↔ DIN 931-1 - replaced by DIN EN 24014 M6 x 30:11
- Angle:147 (0 deg): DIN 931-1 - replaced by DIN EN 24014 M6 x 30:4 ↔ DIN 931-1 - replaced by DIN EN 24014 M6 x 30:11
- Angle:148 (0 deg): DIN 931-1 - replaced by DIN EN 24014 M6 x 30:5 ↔ DIN 931-1 - replaced by DIN EN 24014 M6 x 30:10
- Angle:150 (0 deg): DIN 931-1 - replaced by DIN EN 24014 M6 x 30:5 ↔ DIN 931-1 - replaced by DIN EN 24014 M6 x 30:15
- Angle:151 (0 deg): DIN 931-1 - replaced by DIN EN 24014 M6 x 30:5 ↔ DIN 931-1 - replaced by DIN EN 24014 M6 x 30:12
- Angle:152 (0 deg): DIN 931-1 - replaced by DIN EN 24014 M6 x 30:12 ↔ DIN 931-1 - replaced by DIN EN 24014 M6 x 30:14
- Angle:153 (0 deg): DIN 931-1 - replaced by DIN EN 24014 M6 x 30:9 ↔ DIN 931-1 - replaced by DIN EN 24014 M6 x 30:12
- Angle:154 (0 deg): Plattform-Unterteil:1 ↔ DIN 981 KM 6:7
- Angle:155 (0 deg): DIN 981 KM 6:3 ↔ DIN 981 KM 6:7
- Angle:156 (0 deg): Plattform-Unterteil:1 ↔ DIN 981 KM 6:6
- Angle:157 (0 deg): DIN 981 KM 6:4 ↔ DIN 981 KM 6:6
- Angle:158 (0 deg): Plattform-Unterteil:1 ↔ DIN 981 KM 6:11
- Angle:159 (0 deg): DIN 981 KM 6:10 ↔ DIN 981 KM 6:11
- Angle:160 (0 deg): DIN 981 KM 6:11 ↔ DIN 981 KM 6:13
- Angle:161 (0 deg): DIN 981 KM 6:12 ↔ DIN 981 KM 6:13
- Angle:162 (0 deg): Plattform-Unterteil:1 ↔ DIN 981 KM 6:9
- Angle:163 (0 deg): DIN 981 KM 6:8 ↔ DIN 981 KM 6:9
- Angle:164 (0 deg): Plattform-Unterteil:1 ↔ DIN 981 KM 6:15
- Angle:165 (0 deg): DIN 981 KM 6:14 ↔ DIN 981 KM 6:15
- Mate:654: DIN 625 SKF- with two RS1 seals SKF 6206-2RS1:1 ↔ Spindel:1
- Mate:655: DIN 711 SKF SKF 51108:1 ↔ Spindel:1
- Mate:656: Spindel:1 ↔ DIN 625 SKF- with two RS1 seals SKF 6005-2RSH:1
- Angle:166 (0 deg): Grundplatte:1 ↔ DIN 931-1 - replaced by DIN EN 24014 M12 x 55:4
- Angle:167 (0 deg): Grundplatte:1 ↔ DIN 931-1 - replaced by DIN EN 24014 M12 x 55:3
- Angle:175 (0 deg): DIN 931-1 - replaced by DIN EN 24014 M8 x 45:1 ↔ DIN 931-1 - replaced by DIN EN 24014 M8 x 45:2
- Mate:657: Loslagertopf:1 ↔ Schutzpuffer:1
- Angle:176 (0 deg): Plattform-Unterteil:1 ↔ DIN 931-1 - replaced by DIN EN 24014 M8 x 50:8
- Angle:177 (0 deg): DIN 931-1 - replaced by DIN EN 24014 M8 x 50:7 ↔ DIN 931-1 - replaced by DIN EN 24014 M8 x 50:8
- Angle:178 (0 deg): DIN 931-1 - replaced by DIN EN 24014 M8 x 50:5 ↔ DIN 931-1 - replaced by DIN EN 24014 M8 x 50:7
- Angle:179 (0 deg): DIN 931-1 - replaced by DIN EN 24014 M8 x 50:6 ↔ DIN 931-1 - replaced by DIN EN 24014 M8 x 50:7
- Angle:180 (0 deg): DIN 931-1 - replaced by DIN EN 24014 M8 x 45:1 ↔ DIN 931-1 - replaced by DIN EN 24014 M8 x 50:6
- Angle:181 (0 deg): DIN 931-1 - replaced by DIN EN 24014 M8 x 45:1 ↔ DIN 931-1 - replaced by DIN EN 24014 M8 x 45:2
- Angle:182 (0 deg): DIN 931-1 - replaced by DIN EN 24014 M8 x 45:1 ↔ DIN 931-1 - replaced by DIN EN 24014 M8 x 45:4
- Angle:183 (0 deg): DIN 931-1 - replaced by DIN EN 24014 M8 x 45:1 ↔ DIN 931-1 - replaced by DIN EN 24014 M8 x 45:3